# Autodesk Inventor assembly: Joiner Piece 1764
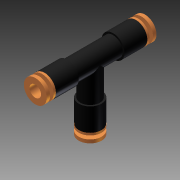
[picture p0: Inventor's stored thumbnail of the model, 180x180]
Saved by Autodesk Inventor 2011 (Build 150239000, 239)
## iProperties
Created: 2010-02-21
Part Number: Joiner Piece 1764
Document SubType Name: Assembly
Designer: jgehrig
Author: jgehrig
## Documents named in this file (3)
- R:\CAD Archives\Pneumatics\Joiner Piece 1764\Joiner Piece 1764.iam
- R:\CAD Archives\Pneumatics\Joiner Piece 1764\Joiner Base 1764.ipt
- R:\CAD Archives\Pneumatics\Joiner Piece 1764\Pneumatic Screw Part 2 1764.ipt
## Components (4 placed, 2 different names)
1. Joiner Base 1764:1 — Insert:1, Insert:2, Insert:3
2. Pneumatic Screw Part 2 1764:1 — Insert:3
3. Pneumatic Screw Part 2 1764:2 — Insert:2
4. Pneumatic Screw Part 2 1764:3 — Insert:1
## Relationships (3: Insert 3)
- Insert:1: Joiner Base 1764:1 ↔ Pneumatic Screw Part 2 1764:3
- Insert:2: Joiner Base 1764:1 ↔ Pneumatic Screw Part 2 1764:2
- Insert:3: Joiner Base 1764:1 ↔ Pneumatic Screw Part 2 1764:1
